# Autodesk Inventor assembly: Assembly1
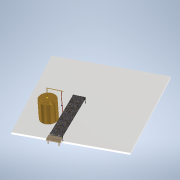
[picture p0: Inventor's stored thumbnail of the model, 180x180]
Saved by Autodesk Inventor 2021 (Build 250183000, 183)
## iProperties
Created: 2021-07-12
Part Number: Assembly1
Document SubType Name: Assembly
Designer: Mahadev Hundarad
Author: Mahadev Hundarad
## Documents named in this file (8)
- C:\Users\Mahadev Hundarad\Desktop\Assembly1.iam
- C:\Users\Mahadev Hundarad\Desktop\motor.ipt
- C:\Users\Mahadev Hundarad\Desktop\belt.ipt
- C:\Users\Mahadev Hundarad\Desktop\base.ipt
- C:\Users\Mahadev Hundarad\Desktop\ee model1620.ipt
- C:\Users\Mahadev Hundarad\Desktop\Part1 containeer.ipt
- C:\Users\Mahadev Hundarad\Desktop\table legs.ipt
- C:\Users\Mahadev Hundarad\Desktop\table top 12062.ipt
## Components (11 placed, 7 different names)
1. motor:1 — Mate:1, Mate:2, Mate:6
2. motor:2 — Mate:3, Mate:4, Mate:5, Mate:7, Mate:8, Mate:9
3. base:1 — Mate:5, Mate:6, Mate:7, Mate:8, Mate:9, Mate:10, Mate:11
4. belt:1 — Mate:1, Mate:2, Mate:3, Mate:4
5. ee model1620:1 — Mate:10, Mate:11, Mate:12
6. Part1 containeer:1 — Mate:12
7. table top 12062:1 — Mate:13, Mate:14, Mate:15, Mate:16, Mate:17, Mate:18, Mate:19, Mate:20
8. table legs:5 — Mate:16, Mate:20
9. table legs:6 — Mate:17, Mate:18
10. table legs:7 — Mate:15, Mate:19
11. table legs:8 — Mate:13, Mate:14
## Relationships (20: Mate 20)
- Mate:1: motor:1 ↔ belt:1
- Mate:2: motor:1 ↔ belt:1
- Mate:3: motor:2 ↔ belt:1
- Mate:4: motor:2 ↔ belt:1
- Mate:5: motor:2 ↔ base:1
- Mate:6: motor:1 ↔ base:1
- Mate:7: motor:2 ↔ base:1
- Mate:8: motor:2 ↔ base:1
- Mate:9: motor:2 ↔ base:1
- Mate:10: base:1 ↔ ee model1620:1
- Mate:11: base:1 ↔ ee model1620:1
- Mate:12: ee model1620:1 ↔ Part1 containeer:1
- Mate:13: table top 12062:1 ↔ table legs:8
- Mate:14: table top 12062:1 ↔ table legs:8
- Mate:15: table top 12062:1 ↔ table legs:7
- Mate:16: table top 12062:1 ↔ table legs:5
- Mate:17: table top 12062:1 ↔ table legs:6
- Mate:18: table top 12062:1 ↔ table legs:6
- Mate:19: table top 12062:1 ↔ table legs:7
- Mate:20: table top 12062:1 ↔ table legs:5
